# Autodesk Inventor assembly: барабан полгый 25-26
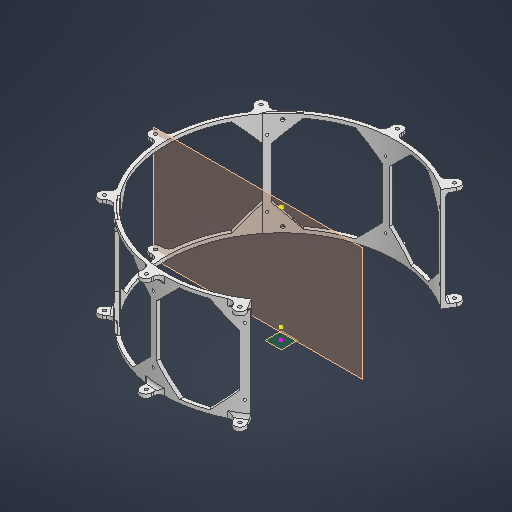
[picture p0: Inventor's stored thumbnail of the model, 512x512]
Saved by Autodesk Inventor 2026.2 (Build 302298000, 298)
## iProperties
Created: 2026-01-06
Part Number: барабан полгый 25-26
Document SubType Name: Assembly
Designer: Phantom
Author: Phantom
## Documents named in this file (4)
- C:\Users\Phantom\Desktop\Phantom16950\барабан полгый 25-26.iam
- C:\Users\Phantom\Desktop\Phantom16950\барабан для портфолио.ipt
- C:\Users\Phantom\Desktop\Phantom16950\барабан для портфолио 2.ipt
- C:\Users\Phantom\Desktop\Phantom16950\барабан для портфолио 3.ipt
## Components (3 placed, 3 different names)
1. барабан для портфолио:1 — Совмещение:1, Совмещение:2, Заподлицо:1, Совмещение:3, Заподлицо:2, Совмещение:4
2. барабан для портфолио 2:1 — Совмещение:1, Совмещение:3, Заподлицо:2
3. барабан для портфолио 3:1 — Совмещение:2, Заподлицо:1, Совмещение:4
## Relationships (6: Mate 4, Flush 2)
- Совмещение:1 [Mate]: барабан для портфолио:1 ↔ барабан для портфолио 2:1
- Совмещение:2 [Mate]: барабан для портфолио:1 ↔ барабан для портфолио 3:1
- Заподлицо:1 [Flush]: барабан для портфолио:1 ↔ барабан для портфолио 3:1
- Совмещение:3 [Mate]: барабан для портфолио:1 ↔ барабан для портфолио 2:1
- Заподлицо:2 [Flush]: барабан для портфолио:1 ↔ барабан для портфолио 2:1
- Совмещение:4 [Mate]: барабан для портфолио:1 ↔ барабан для портфолио 3:1
